# Autodesk Inventor assembly: WheelAssembly3.0
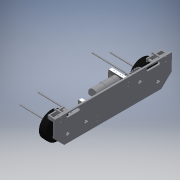
[picture p0: Inventor's stored thumbnail of the model, 180x180]
Saved by Autodesk Inventor 2017 (Build 210142000, 142)
## iProperties
Created: 2017-07-22
Part Number: WheelAssembly3.0
Document SubType Name: Assembly
Designer: User
Author: User
## Documents named in this file (14)
- C:\Robotics\CAD\WheelAssembly3.0.iam
- C:\Robotics\CAD\2016-17_CAD\DriveTrain\DriveTrain3.0.ipt
- C:\Robotics\CAD\COTSParts\Motors\Andymark 2964  NeveRest 40 Motor.ipt
- C:\Robotics\CAD\COTSParts\Tetrix\tetrix-motor-mounts-1.snapshot.1\Tetrex 2pc motor mount.ipt
- C:\Robotics\CAD\COTSParts\Actobotics\615 parts\615398.ipt
- C:\Robotics\CAD\2016-17_CAD\Custom COTS\4inax.ipt
- C:\Robotics\CAD\COTSParts\Actobotics\615 parts\615106.ipt
- C:\Robotics\CAD\COTSParts\Actobotics\545 parts\545556.ipt
- C:\Robotics\CAD\COTSParts\Actobotics\615 parts\615114.ipt
- C:\Robotics\CAD\2016-17_CAD\DriveTrain\Tensioner.iam
- C:\Robotics\CAD\COTSParts\Actobotics\545 parts\545456.ipt
- C:\Robotics\CAD\COTSParts\Wheels\4in Wheel Intergreated Hub 8mm Rev2.ipt
- C:\Robotics\CAD\2016-17_CAD\DriveTrain\MotorFixedPositionMount.ipt
- C:\Robotics\CAD\COTSParts\Actobotics\Thrust Bearings\6655K13.ipt
## Components (36 placed, 13 different names)
1. DriveTrain3.0:1 — Flush:3, Flush:4, Mate:2, Flush:5, Mate:3, Flush:6, Angle:1, Insert:7, Insert:8, Angle:2, Insert:9, Insert:10, Insert:16, Insert:17, Flush:17, Flush:18, Mate:21, Flush:19, Mate:22, Flush:20
2. Andymark 2964  NeveRest 40 Motor:1 — Insert:3, Insert:6, Angle:2
3. Andymark 2964  NeveRest 40 Motor:2 — Insert:4, Insert:5, Angle:1
4. Tetrex 2pc motor mount:1 — Insert:3, Flush:3, Mate:3, Flush:6, Mate:17, Insert:45, Insert:46
5. Tetrex 2pc motor mount:2 — Insert:4, Flush:4, Mate:2, Flush:5, Mate:10, Insert:30, Insert:31
6. 615398:1 — Insert:5, Insert:44
7. 615398:2 — Insert:6
8. 615398:3 — Insert:7, Insert:36
9. 615398:4 — Insert:8, Insert:38
10. 4inax:1 — Insert:9, Mate:18
11. 4inax:2 — Insert:10, Mate:8, Mate:16, Mate:19, Mate:23
12. 615106:2 — Insert:26, Flush:21
13. 4inax:3 — Insert:16
14. 4inax:4 — Insert:17, Mate:9, Mate:14, Mate:15
15. 545556:3 — Insert:26, Mate:14, Insert:29
16. 615114:2 — Insert:37, Flush:21
17. 545556:4 — Insert:36, Insert:37, Insert:43
18. Tensioner:1 [sub-assembly] — Flush:17, Flush:18, Mate:21
19. 545556:5 — Mate:23, Mate:24, Insert:40
20. 545456:1 — Insert:40, Insert:41
21. 4in Wheel Intergreated Hub 8mm Rev2:1 — Insert:41
22. DriveTrain3.0:2 — Mate:8, Mate:9, Mate:10
23. Tensioner:2 [sub-assembly] — Flush:19, Mate:22, Flush:20
24. 545556:6 — Insert:27, Insert:29
25. 545456:2 — Insert:27, Insert:28
26. 4in Wheel Intergreated Hub 8mm Rev2:2 — Insert:28
27. DriveTrain3.0:3 — Mate:15, Mate:16, Mate:17
28. MotorFixedPositionMount:1 — Insert:30, Insert:31
29. MotorFixedPositionMount:2 — Insert:45, Insert:46
30. 545556:7 — Mate:18, Insert:38, Insert:39, Insert:42
31. 545556:8 — Insert:35, Mate:19
32. 615114:3 — Insert:39, Flush:22
33. 615106:3 — Insert:35, Flush:22, Mate:24
34. 6655K13:1 — Insert:42
35. 6655K13:2 — Insert:43
36. 6655K13:3 — Insert:44
## Relationships (55: Insert 28, Mate 15, Flush 10, Angle 2)
- Insert:3: Andymark 2964  NeveRest 40 Motor:1 ↔ Tetrex 2pc motor mount:1
- Insert:4: Andymark 2964  NeveRest 40 Motor:2 ↔ Tetrex 2pc motor mount:2
- Flush:3 (159.5374 mm): DriveTrain3.0:1 ↔ Tetrex 2pc motor mount:1
- Flush:4 (159.5374 mm): DriveTrain3.0:1 ↔ Tetrex 2pc motor mount:2
- Insert:5: Andymark 2964  NeveRest 40 Motor:2 ↔ 615398:1
- Mate:2: DriveTrain3.0:1 ↔ Tetrex 2pc motor mount:2
- Flush:5 (7.3152 mm): DriveTrain3.0:1 ↔ Tetrex 2pc motor mount:2
- Mate:3: DriveTrain3.0:1 ↔ Tetrex 2pc motor mount:1
- Flush:6 (-20.3454 mm): DriveTrain3.0:1 ↔ Tetrex 2pc motor mount:1
- Angle:1 (0 deg): DriveTrain3.0:1 ↔ Andymark 2964  NeveRest 40 Motor:2
- Insert:6: Andymark 2964  NeveRest 40 Motor:1 ↔ 615398:2
- Insert:7 (25.4508 mm): DriveTrain3.0:1 ↔ 615398:3
- Insert:8 (25.4508 mm): DriveTrain3.0:1 ↔ 615398:4
- Angle:2 (180 deg): DriveTrain3.0:1 ↔ Andymark 2964  NeveRest 40 Motor:1
- Insert:9 (-6.35 mm): DriveTrain3.0:1 ↔ 4inax:1
- Insert:10 (-6.35 mm): DriveTrain3.0:1 ↔ 4inax:2
- Insert:16 (-6.35 mm): DriveTrain3.0:1 ↔ 4inax:3
- Insert:17 (-6.35 mm): DriveTrain3.0:1 ↔ 4inax:4
- Mate:8: 4inax:2 ↔ DriveTrain3.0:2
- Mate:9: 4inax:4 ↔ DriveTrain3.0:2
- Mate:10: Tetrex 2pc motor mount:2 ↔ DriveTrain3.0:2
- Insert:26: 615106:2 ↔ 545556:3
- Mate:14: 4inax:4 ↔ 545556:3
- Insert:27: 545556:6 ↔ 545456:2
- Insert:28: 545456:2 ↔ 4in Wheel Intergreated Hub 8mm Rev2:2
- Insert:29 (3.175 mm): 545556:3 ↔ 545556:6
- Mate:15: 4inax:4 ↔ DriveTrain3.0:3
- Mate:16: 4inax:2 ↔ DriveTrain3.0:3
- Mate:17: Tetrex 2pc motor mount:1 ↔ DriveTrain3.0:3
- Insert:30: Tetrex 2pc motor mount:2 ↔ MotorFixedPositionMount:1
- Insert:31: Tetrex 2pc motor mount:2 ↔ MotorFixedPositionMount:1
- Insert:35: 545556:8 ↔ 615106:3
- Mate:18: 4inax:1 ↔ 545556:7
- Mate:19: 4inax:2 ↔ 545556:8
- Flush:17: DriveTrain3.0:1 ↔ Tensioner:1
- Flush:18 (34.925 mm): DriveTrain3.0:1 ↔ Tensioner:1
- Mate:21: DriveTrain3.0:1 ↔ Tensioner:1
- Flush:19: DriveTrain3.0:1 ↔ Tensioner:2
- Mate:22: DriveTrain3.0:1 ↔ Tensioner:2
- Flush:20 (-34.925 mm): DriveTrain3.0:1 ↔ Tensioner:2
- Insert:36: 615398:3 ↔ 545556:4
- Insert:37: 615114:2 ↔ 545556:4
- Flush:21: 615106:2 ↔ 615114:2
- Insert:38: 615398:4 ↔ 545556:7
- Insert:39: 545556:7 ↔ 615114:3
- Flush:22: 615114:3 ↔ 615106:3
- Mate:23: 4inax:2 ↔ 545556:5
- Mate:24 (3.175 mm): 545556:5 ↔ 615106:3
- Insert:40: 545556:5 ↔ 545456:1
- Insert:41: 545456:1 ↔ 4in Wheel Intergreated Hub 8mm Rev2:1
- Insert:42: 545556:7 ↔ 6655K13:1
- Insert:43: 545556:4 ↔ 6655K13:2
- Insert:44: 615398:1 ↔ 6655K13:3
- Insert:45: Tetrex 2pc motor mount:1 ↔ MotorFixedPositionMount:2
- Insert:46: Tetrex 2pc motor mount:1 ↔ MotorFixedPositionMount:2
